# Autodesk Inventor assembly: X-Yconfig
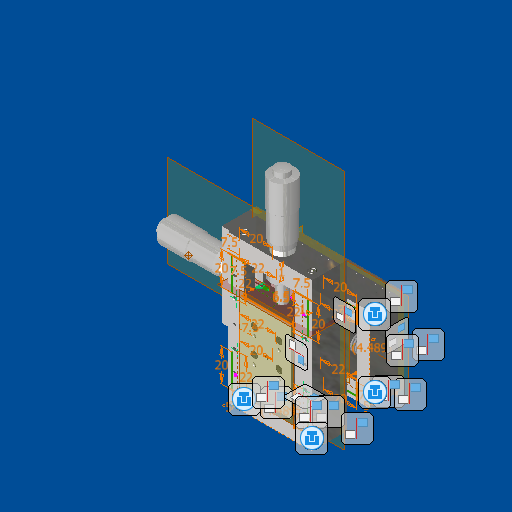
[picture p0: Inventor's stored thumbnail of the model, 512x512]
Saved by Autodesk Inventor 2025.1 (Build 291241000, 241)
## iProperties
Created: 2025-02-04
Part Number: X-Yconfig
Document SubType Name: Assembly
Designer: konch
Author: konch
## Documents named in this file (3)
- C:\Users\konch\OneDrive\Desktop\FMD_Konrad_Kosuge\X-Yconfig.iam
- C:\Users\konch\OneDrive\Desktop\FMD_Konrad_Kosuge\PLA_Konrad_Kosugesnapshot7.iam
- C:\Users\konch\OneDrive\Documents\Inventor\Content Center Files\R2025\en-US\ISO 4762(2)\ISO 4762 - M3 x 8ISO.ipt
## Components (6 placed, 2 different names)
1. PLA_Konrad_Kosugesnapshot7:1 [sub-assembly] — Mate:1, Mate:2, Mate:3
2. PLA_Konrad_Kosugesnapshot7:2 [sub-assembly] — Mate:1, Mate:2, Mate:3, Rotational:1, Rotational:2, Rotational:3, Rotational:4
3. ISO 4762 M3 x 8:1 — Rotational:2
4. ISO 4762 M3 x 8:2 — Rotational:3
5. ISO 4762 M3 x 8:4 — Rotational:1
6. ISO 4762 M3 x 8:5 — Rotational:4
## Relationships (7: RevoluteJoint 4, Mate 3)
- Mate:1: PLA_Konrad_Kosugesnapshot7:1 ↔ PLA_Konrad_Kosugesnapshot7:2
- Mate:2: PLA_Konrad_Kosugesnapshot7:1 ↔ PLA_Konrad_Kosugesnapshot7:2
- Mate:3: PLA_Konrad_Kosugesnapshot7:1 ↔ PLA_Konrad_Kosugesnapshot7:2
- Rotational:1 [RevoluteJoint]: PLA_Konrad_Kosugesnapshot7:2 ↔ ISO 4762 M3 x 8:4
- Rotational:2 [RevoluteJoint]: PLA_Konrad_Kosugesnapshot7:2 ↔ ISO 4762 M3 x 8:1
- Rotational:3 [RevoluteJoint]: PLA_Konrad_Kosugesnapshot7:2 ↔ ISO 4762 M3 x 8:2
- Rotational:4 [RevoluteJoint]: PLA_Konrad_Kosugesnapshot7:2 ↔ ISO 4762 M3 x 8:5
